# Autodesk Inventor assembly: Tracker
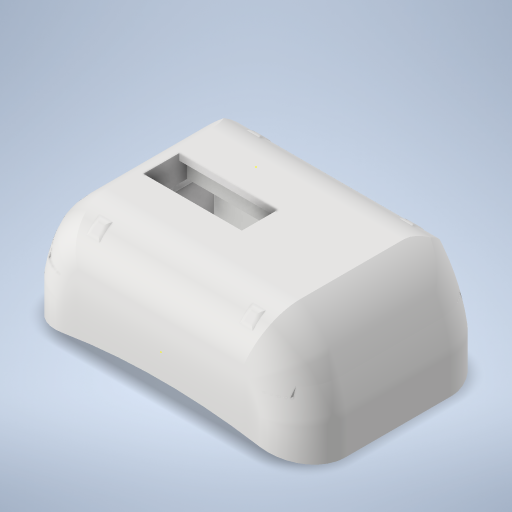
[picture p0: Inventor's stored thumbnail of the model, 512x512]
Saved by Autodesk Inventor 2023 (Build 270158000, 158)
## iProperties
Created: 2022-06-04
Part Number: Tracker
Document SubType Name: Assembly
Designer: tianyu
Author: tianyu
## Documents named in this file (3)
- C:\Users\bit86\Desktop\Working\Inventer\Tracker.iam
- C:\Users\bit86\Desktop\Working\Inventer\Enclosure-Top.ipt
- C:\Users\bit86\Desktop\Working\Inventer\Enclosure-Base.ipt
## Components (2 placed, 2 different names)
1. Enclosure-Base:1 — Mate:1, Mate:2, Mate:3
2. Enclosure-Top:1 — Mate:1, Mate:2, Mate:3
## Relationships (3: Mate 3)
- Mate:1: Enclosure-Base:1 ↔ Enclosure-Top:1
- Mate:2: Enclosure-Base:1 ↔ Enclosure-Top:1
- Mate:3: Enclosure-Base:1 ↔ Enclosure-Top:1
